# Autodesk Inventor assembly: gimbal
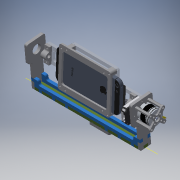
[picture p0: Inventor's stored thumbnail of the model, 180x180]
Saved by Autodesk Inventor 2016 (Build 200138000, 138)
## iProperties
Created: 2015-12-01
Part Number: gimbal
Document SubType Name: Assembly
Designer: jufranz
Author: jufranz
## Documents named in this file (4)
- C:\Users\jfranz\Documents\GitHub\perspection\hardware\cad\gimbal.iam
- C:\Users\jfranz\Documents\GitHub\perspection\hardware\cad\yaw-frame.iam
- C:\Users\jfranz\Documents\GitHub\perspection\hardware\cad\pitch-frame.iam
- C:\Users\jfranz\Documents\GitHub\perspection\hardware\cad\hex_plate.ipt
## Components (3 placed, 3 different names)
1. yaw-frame:1 [sub-assembly] — Insert:1, Mate:1, Flush:1
2. pitch-frame:1 [sub-assembly] — Insert:1
3. hex_plate:1 — Mate:1, Flush:1
## Relationships (3: Insert 1, Mate 1, Flush 1)
- Insert:1 (-12 mm): yaw-frame:1 ↔ pitch-frame:1
- Mate:1: yaw-frame:1 ↔ hex_plate:1
- Flush:1: yaw-frame:1 ↔ hex_plate:1
